# Autodesk Inventor assembly: Assemblage
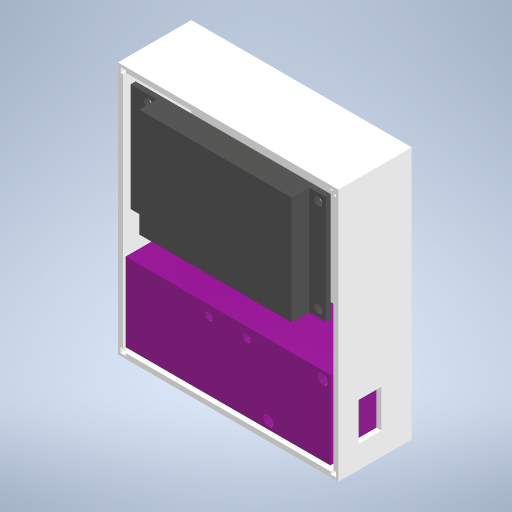
[picture p0: Inventor's stored thumbnail of the model, 512x512]
Saved by Autodesk Inventor 2023 (Build 270158000, 158)
## iProperties
Created: 2023-04-14
Part Number: Assemblage
Document SubType Name: Assembly
Designer: Timothée
Author: Timothée
## Documents named in this file (5)
- C:\Users\timot\Documents\Workspace\ELEC_NUM\EON-NUM\Ressources\Project case\Assemblage.iam
- C:\Users\timot\Documents\Workspace\ELEC_NUM\EON-NUM\Ressources\Project case\Ecran.ipt
- C:\Users\timot\Documents\Workspace\ELEC_NUM\EON-NUM\Ressources\Project case\Bluepill.ipt
- C:\Users\timot\Documents\Files\3D\Case.ipt
- C:\Users\timot\Documents\Files\3D\MainCase.ipt
## Components (4 placed, 4 different names)
1. Ecran:1 — Flush:1, Mate:1, Mate:2
2. Bluepill:1 — Mate:3, Flush:2, Flush:3
3. Case:1 — Flush:1, Mate:1, Mate:2, Mate:3, Flush:2, Flush:3, Flush:4
4. MainCase:1 — Flush:4
## Relationships (7: Flush 4, Mate 3)
- Flush:1 (-4 mm): Ecran:1 ↔ Case:1
- Mate:1: Ecran:1 ↔ Case:1
- Mate:2: Ecran:1 ↔ Case:1
- Mate:3: Bluepill:1 ↔ Case:1
- Flush:2 (3 mm): Bluepill:1 ↔ Case:1
- Flush:3 (4 mm): Bluepill:1 ↔ Case:1
- Flush:4: Case:1 ↔ MainCase:1
